# Autodesk Inventor assembly: Shoulder
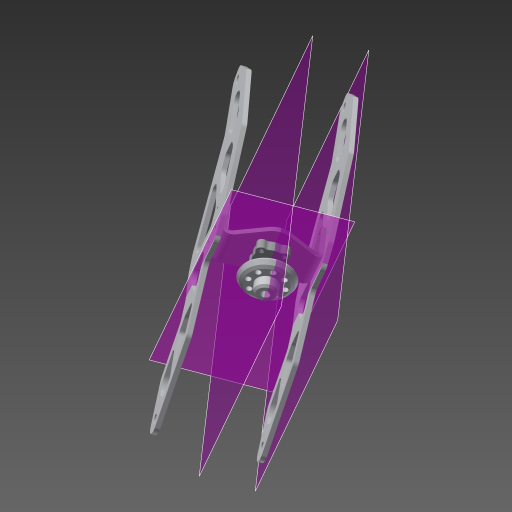
[picture p0: Inventor's stored thumbnail of the model, 512x512]
Saved by Autodesk Inventor 2023 (Build 270158000, 158)
## iProperties
Created: 2020-03-24
Part Number: Shoulder
Document SubType Name: Assembly
Designer: valer
Mass: 4853.13 g
Surface Area: 3141.52 cm^2
Volume: 1403.99 cm^3
Density: 3.45667 g/cm^3
Author: valer
## Documents named in this file (6)
- C:\Users\Val\Desktop\drummingrobot\src\parts\export\Shoulder.iam
- C:\Users\Val\Desktop\drummingrobot\src\parts\UpperArmBracket.ipt
- C:\Users\Val\Desktop\drummingrobot\src\parts\UpperArmBracketBase.ipt
- C:\Users\Val\Desktop\drummingrobot\src\parts\external\ShoulderMiterGear.ipt
- C:\Users\Val\Desktop\drummingrobot\src\parts\external\ServoShaft.ipt
- C:\Users\Val\Desktop\drummingrobot\src\parts\external\Shoulder6mmDShaftHub-545578.ipt
## Components (7 placed, 5 different names)
1. UpperArmBracket:5 — Mate:376, Mate:378, Mate:379, Flush:4
2. UpperArmBracket:6 — Mate:377, Mate:380, Mate:381, Angle:1
3. ShoulderMiterGear:2 — Mate:382, Flush:2
4. ShoulderServoShaft:2 — Mate:374, Mate:382, Flush:1
5. UpperArmBracketBase:1 — Mate:371, Mate:372, Mate:373, Mate:376, Mate:377, Mate:378, Mate:379, Mate:380, Mate:381, Flush:2, Mate:383, Mate:384, Flush:5, Mate:385, Angle:2
6. Shoulder6mmDShaftHub-545578:1 — Mate:371, Mate:372, Mate:373, Mate:374, Flush:1, Flush:3
7. Shoulder6mmDShaftHub-545578:2 — Flush:5, Mate:385, Angle:2
## Relationships (21: Mate 14, Flush 5, Angle 2)
- Mate:371: UpperArmBracketBase:1 ↔ Shoulder6mmDShaftHub-545578:1
- Mate:372: UpperArmBracketBase:1 ↔ Shoulder6mmDShaftHub-545578:1
- Mate:373: UpperArmBracketBase:1 ↔ Shoulder6mmDShaftHub-545578:1
- Mate:374: ShoulderServoShaft:2 ↔ Shoulder6mmDShaftHub-545578:1
- Mate:376: UpperArmBracket:5 ↔ UpperArmBracketBase:1
- Mate:377: UpperArmBracket:6 ↔ UpperArmBracketBase:1
- Mate:378: UpperArmBracket:5 ↔ UpperArmBracketBase:1
- Mate:379: UpperArmBracket:5 ↔ UpperArmBracketBase:1
- Mate:380: UpperArmBracket:6 ↔ UpperArmBracketBase:1
- Mate:381: UpperArmBracket:6 ↔ UpperArmBracketBase:1
- Mate:382: ShoulderMiterGear:2 ↔ ShoulderServoShaft:2
- Flush:1 (-4 mm): ShoulderServoShaft:2 ↔ Shoulder6mmDShaftHub-545578:1
- Flush:2 (-21.1582 mm): ShoulderMiterGear:2 ↔ UpperArmBracketBase:1
- Flush:3: Shoulder6mmDShaftHub-545578:1
- Mate:383: UpperArmBracketBase:1
- Mate:384: UpperArmBracketBase:1
- Angle:1 (0 deg): UpperArmBracket:6
- Flush:4: UpperArmBracket:5
- Flush:5: UpperArmBracketBase:1 ↔ Shoulder6mmDShaftHub-545578:2
- Mate:385: UpperArmBracketBase:1 ↔ Shoulder6mmDShaftHub-545578:2
- Angle:2 (180 deg): UpperArmBracketBase:1 ↔ Shoulder6mmDShaftHub-545578:2
